# Autodesk Inventor assembly: TOOLHEAD_TO_GRABBER
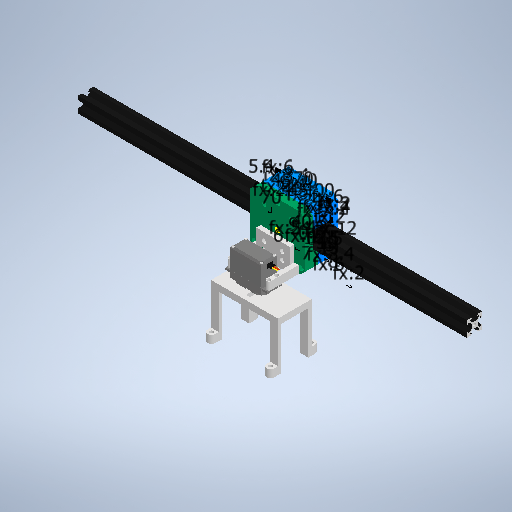
[picture p0: Inventor's stored thumbnail of the model, 512x512]
Saved by Autodesk Inventor 2025.1 (Build 291241000, 241)
## iProperties
Created: 2024-11-04
Part Number: TOOLHEAD_TO_GRABBER
Document SubType Name: Assembly
Designer: m_kni
Author: m_kni
## Documents named in this file (5)
- C:\Users\m_kni\OneDrive\Documents\GitHub\Perovskite-Automated-Synthesis-System\CAD\Gripper\TOOLHEAD_TO_GRABBER.iam
- C:\Users\m_kni\OneDrive\Documents\GitHub\Perovskite-Automated-Synthesis-System\CAD\Gantry\Toolhead\Toolhead.iam
- C:\Users\m_kni\OneDrive\Documents\GitHub\Perovskite-Automated-Synthesis-System\CAD\Gripper\SERVO_TO_TOOLHEAD.ipt
- C:\Users\m_kni\OneDrive\Documents\GitHub\Perovskite-Automated-Synthesis-System\CAD\Non 3D Printed Parts\Motors and Servos\Servo MG996R.ipt
- C:\Users\m_kni\OneDrive\Documents\GitHub\Perovskite-Automated-Synthesis-System\CAD\Gripper\ATTACHMENT_TOOLHEAD_GRIPPER.ipt
## Components (4 placed, 4 different names)
1. Toolhead:1 [sub-assembly] — Insert:1
2. SERVO_TO_TOOLHEAD:1 — Insert:1, Insert:2
3. Servo MG996R:1 — Insert:2, Insert:3, Angle:1
4. ATTACHMENT_TOOLHEAD_GRIPPER:1 — Insert:3, Angle:1
## Relationships (4: Insert 3, Angle 1)
- Insert:1: Toolhead:1 ↔ SERVO_TO_TOOLHEAD:1
- Insert:2: SERVO_TO_TOOLHEAD:1 ↔ Servo MG996R:1
- Insert:3: Servo MG996R:1 ↔ ATTACHMENT_TOOLHEAD_GRIPPER:1
- Angle:1 (0 deg): Servo MG996R:1 ↔ ATTACHMENT_TOOLHEAD_GRIPPER:1
